# Autodesk Inventor assembly: ModuloEsquinero
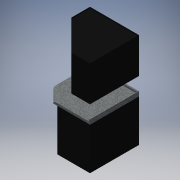
[picture p0: Inventor's stored thumbnail of the model, 180x180]
Saved by Autodesk Inventor 2016 (Build 200138000, 138)
## iProperties
Created: 2015-11-25
Part Number: ModuloEsquinero
Document SubType Name: Assembly
Designer: Daniela
Author: Daniela
## Documents named in this file (3)
- D:\Documents\Carrera\11.Semeste_II_2015\Computacion_grafica\Proyecto\COCINA_FINAL\Cocina\ModuloEsquinero.iam
- D:\Documents\Carrera\11.Semeste_II_2015\Computacion_grafica\Proyecto\COCINA_FINAL\Cocina\esquinero.ipt
- D:\Documents\Carrera\11.Semeste_II_2015\Computacion_grafica\Proyecto\COCINA_FINAL\Cocina\meson_esquinero.ipt
## Components (2 placed, 2 different names)
1. esquinero:1 — Mate:1, Flush:1, Flush:2
2. meson_esquinero:1 — Mate:1, Flush:1, Flush:2
## Relationships (3: Flush 2, Mate 1)
- Mate:1: esquinero:1 ↔ meson_esquinero:1
- Flush:1: esquinero:1 ↔ meson_esquinero:1
- Flush:2: esquinero:1 ↔ meson_esquinero:1
